# Autodesk Inventor assembly: THREAD ASSEMBLY
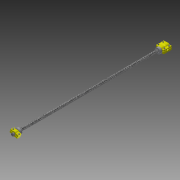
[picture p0: Inventor's stored thumbnail of the model, 180x180]
Saved by Autodesk Inventor 2013 (Build 170138000, 138)
## iProperties
Created: 2013-12-04
Part Number: THREAD ASSEMBLY
Document SubType Name: Assembly
Designer: employee
Author: employee
## Documents named in this file (7)
- C:\Users\employee\Desktop\ConceptFORGE\ConceptFORGE\LISA Simpson\INVENTOR FILES\THREAD ASSEMBLY.iam
- C:\Users\employee\Desktop\ConceptFORGE\ConceptFORGE\LISA Simpson\INVENTOR FILES\COUPLER.ipt
- C:\Users\employee\Desktop\ConceptFORGE\ConceptFORGE\LISA Simpson\INVENTOR FILES\7_16 TORQSPLINE.ipt
- C:\Users\employee\Desktop\ConceptFORGE\ConceptFORGE\LISA Simpson\INVENTOR FILES\_1607.ipt
- C:\Users\employee\Desktop\ConceptFORGE\ConceptFORGE\LISA Simpson\INVENTOR FILES\THREAD CLAMP.ipt
- C:\Users\employee\Desktop\ConceptFORGE\ConceptFORGE\LISA Simpson\INVENTOR FILES\M3 NUT.ipt
- C:\Users\employee\Desktop\ConceptFORGE\ConceptFORGE\LISA Simpson\INVENTOR FILES\M3x16.ipt
## Components (17 placed, 6 different names)
1. COUPLER:1 — Mate:3, Insert:4, Insert:5, Insert:7, Insert:8, Angle:1, Angle:2, Angle:3, Insert:9
2. 7_16 TORQSPLINE:1 — Mate:3
3. _1607:1 — Insert:10, Mate:6, Mate:7
4. _1607:2 — Insert:9, Mate:6, Mate:7
5. THREAD CLAMP:1 — Insert:3, Insert:6, Angle:3, Angle:4, Insert:10
6. M3 NUT:2 — Insert:6, Angle:4
7. M3x16:3 — Insert:3
8. M3x16:2 — Insert:5
9. M3 NUT:1 — Insert:7, Angle:1
10. M3 NUT:3 — Insert:8, Angle:2
11. M3x16:1 — Insert:4
12. M3 NUT:4
13. M3x16:4
14. M3x16:5
15. M3 NUT:5
16. M3 NUT:6
17. M3x16:6
## Component patterns: (2 elements, first: M3 NUT:2 + M3x16:3 + M3x16:2 + M3 NUT:1 + M3 NUT:3 + M3x16:1)
## Relationships (15: Insert 8, Angle 4, Mate 3)
- Mate:3: COUPLER:1 ↔ 7_16 TORQSPLINE:1
- Insert:3: THREAD CLAMP:1 ↔ M3x16:3
- Insert:4: COUPLER:1 ↔ M3x16:1
- Insert:5: COUPLER:1 ↔ M3x16:2
- Insert:6: THREAD CLAMP:1 ↔ M3 NUT:2
- Insert:7: COUPLER:1 ↔ M3 NUT:1
- Insert:8: COUPLER:1 ↔ M3 NUT:3
- Angle:1 (0 deg): COUPLER:1 ↔ M3 NUT:1
- Angle:2 (0 deg): COUPLER:1 ↔ M3 NUT:3
- Angle:3 (21.58 deg): COUPLER:1 ↔ THREAD CLAMP:1
- Angle:4 (0 deg): THREAD CLAMP:1 ↔ M3 NUT:2
- Insert:9: COUPLER:1 ↔ _1607:2
- Insert:10: _1607:1 ↔ THREAD CLAMP:1
- Mate:6: _1607:1 ↔ _1607:2
- Mate:7 (-577.4436 mm): _1607:1 ↔ _1607:2
